# Autodesk Inventor assembly: Beamerscope_r2
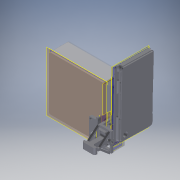
[picture p0: Inventor's stored thumbnail of the model, 180x180]
Saved by Autodesk Inventor 2016 (Build 200138000, 138)
## iProperties
Created: 2016-09-10
Part Number: Beamerscope_r2
Material: Generisch
Document SubType Name: Assembly
Designer: Bene
Mass: 220.683 g
Surface Area: 1737.49 cm^2
Volume: 289.423 cm^3
Density: 0.762493 g/cm^3
Author: Bene
## Documents named in this file (15)
- C:\Users\Bene\Dropbox\Dokumente\OpticalDesign\Beamerscope\Inventor\Beamerscope_r2\Beamerscope_r2.iam
- C:\Users\Bene\Dropbox\Dokumente\OpticalDesign\Beamerscope\Inventor\Beamerscope_r2\01_Beamer_Gehäuse.ipt
- C:\Users\Bene\Dropbox\Dokumente\OpticalDesign\Beamerscope\Inventor\Beamerscope_r2\02_Beamer_Deckel.ipt
- C:\Users\Bene\Dropbox\Dokumente\OpticalDesign\Beamerscope\Inventor\Beamerscope_r2\Lenstube.iam
- C:\Users\Bene\Dropbox\Dokumente\OpticalDesign\Beamerscope\Inventor\Beamerscope_r2\03_Tubeholder_bottom.ipt
- C:\Users\Bene\Dropbox\Dokumente\OpticalDesign\Beamerscope\Inventor\Beamerscope_r2\04_Tubeholder_top.ipt
- C:\Users\Bene\Dropbox\Dokumente\OpticalDesign\Beamerscope\Inventor\Beamerscope_r2\10_Mikrolinse.ipt
- C:\Users\Bene\Dropbox\Dokumente\OpticalDesign\Beamerscope\Inventor\Beamerscope_r2\11_Objektträger.ipt
- C:\Users\Bene\Dropbox\Dokumente\OpticalDesign\Beamerscope\Inventor\Beamerscope_r2\20_Z-Focus.ipt
- C:\Users\Bene\Dropbox\Dokumente\OpticalDesign\Beamerscope\Inventor\Beamerscope_r2\21_Connection_Projector_Focus.ipt
- C:\Users\Bene\Dropbox\Dokumente\OpticalDesign\Beamerscope\Inventor\Beamerscope_r2\31_Handyaufnahme_2.ipt
- C:\Users\Bene\Dropbox\Dokumente\OpticalDesign\Beamerscope\Inventor\Beamerscope_r2\31_Handyaufnahme_3.ipt
- C:\Users\Bene\Dropbox\Dokumente\OpticalDesign\Beamerscope\Inventor\Beamerscope_r2\00_SonyXperiaZ3correct.ipt
- C:\Users\Bene\Dropbox\Dokumente\OpticalDesign\Beamerscope\Inventor\Beamerscope_r2\32_Handycase.ipt
- C:\Users\Bene\Dropbox\Dokumente\OpticalDesign\Beamerscope\Inventor\Beamerscope_r2\22_Focus_Objectadapter.ipt
## Components (14 placed, 14 different names)
1. 01_Beamer_Gehäuse:1 — Fluchtend:1, Passend:3, Passend:4, Fluchtend:2, Fluchtend:3, Fluchtend:7, Fluchtend:8, Passend:6, Passend:7, Passend:8
2. 02_Beamer_Deckel:1 — Fluchtend:1
3. Lenstube:1 [sub-assembly] — Passend:3, Passend:4
4. 03_Tubeholder_bottom:1 — Fluchtend:2, Fluchtend:3
5. 04_Tubeholder_top:1
6. 10_Mikrolinse:1 — Passend:5
7. 11_Objektträger:1 — Passend:5
8. 20_Z-Focus:1 — Fluchtend:9, Fluchtend:11
9. 21_Connection_Projector_Focus:1 — Fluchtend:7, Fluchtend:8, Fluchtend:9
10. 31_Handyaufnahme_2:1 — Fluchtend:10, Einfügen:1, Einfügen:2, Passend:9
11. 31_Handyaufnahme_3:1 — Passend:6, Passend:7, Passend:8, Passend:9
12. 00_SonyXperiaZ3correct:1 — Fluchtend:10
13. 32_Handycase:1 — Einfügen:1, Einfügen:2
14. 22_Focus_Objectadapter:1 — Fluchtend:11
## Relationships (17: Flush 8, Mate 7, Insert 2)
- Fluchtend:1 [Flush]: 01_Beamer_Gehäuse:1 ↔ 02_Beamer_Deckel:1
- Passend:3 [Mate] (22.5 mm): 01_Beamer_Gehäuse:1 ↔ Lenstube:1
- Passend:4 [Mate]: 01_Beamer_Gehäuse:1 ↔ Lenstube:1
- Fluchtend:2 [Flush]: 01_Beamer_Gehäuse:1 ↔ 03_Tubeholder_bottom:1
- Fluchtend:3 [Flush]: 01_Beamer_Gehäuse:1 ↔ 03_Tubeholder_bottom:1
- Passend:5 [Mate]: 10_Mikrolinse:1 ↔ 11_Objektträger:1
- Fluchtend:7 [Flush]: 01_Beamer_Gehäuse:1 ↔ 21_Connection_Projector_Focus:1
- Fluchtend:8 [Flush]: 01_Beamer_Gehäuse:1 ↔ 21_Connection_Projector_Focus:1
- Fluchtend:9 [Flush]: 20_Z-Focus:1 ↔ 21_Connection_Projector_Focus:1
- Passend:6 [Mate]: 01_Beamer_Gehäuse:1 ↔ 31_Handyaufnahme_3:1
- Passend:7 [Mate]: 01_Beamer_Gehäuse:1 ↔ 31_Handyaufnahme_3:1
- Passend:8 [Mate]: 01_Beamer_Gehäuse:1 ↔ 31_Handyaufnahme_3:1
- Fluchtend:10 [Flush]: 31_Handyaufnahme_2:1 ↔ 00_SonyXperiaZ3correct:1
- Einfügen:1 [Insert] (-2 mm): 31_Handyaufnahme_2:1 ↔ 32_Handycase:1
- Einfügen:2 [Insert]: 31_Handyaufnahme_2:1 ↔ 32_Handycase:1
- Passend:9 [Mate]: 31_Handyaufnahme_2:1 ↔ 31_Handyaufnahme_3:1
- Fluchtend:11 [Flush]: 20_Z-Focus:1 ↔ 22_Focus_Objectadapter:1
